# Autodesk Inventor assembly: Крейцкопфф
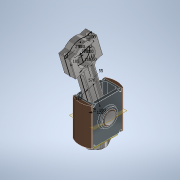
[picture p0: Inventor's stored thumbnail of the model, 180x180]
Saved by Autodesk Inventor 2021 (Build 250183000, 183)
## iProperties
Created: 2020-11-30
Part Number: Крейцкопфф
Document SubType Name: Assembly
Designer: Тимоха
Author: Тимоха
## Documents named in this file (17)
- C:\Users\Тимоха\Desktop\КР Компрессор\compressor\Крейцкопфф.iam
- C:\Users\Тимоха\Desktop\КР Компрессор\compressor\Втулка палец шатун.ipt
- C:\Users\Тимоха\Desktop\КР Компрессор\compressor\Втулка под палец.ipt
- C:\Users\Тимоха\Desktop\КР Компрессор\compressor\Крейцкопф.ipt
- C:\Users\Тимоха\Desktop\КР Компрессор\compressor\Шатун.ipt
- C:\Users\Тимоха\Desktop\КР Компрессор\compressor\Втулка под палец_MIR.ipt
- C:\Users\Тимоха\Desktop\КР Компрессор\compressor\Палец.ipt
- C:\Users\Тимоха\Desktop\КР Компрессор\compressor\Фланецгайка.ipt
- C:\Users\Тимоха\Desktop\КР Компрессор\compressor\Башмак.ipt
- C:\Users\Тимоха\Desktop\КР Компрессор\compressor\Башмак_MIR.ipt
- C:\Users\Тимоха\Desktop\КР Компрессор\compressor\Гайка шток.ipt
- C:\Users\Тимоха\Desktop\КР Компрессор\compressor\Прокладка крейцкопф.ipt
- C:\Users\Тимоха\Documents\Inventor\Content Center Files\R2021\ru-RU\GOST 8878-93\Винт M6-6gx25 ГОСТ 8878-93.ipt
- C:\Users\Тимоха\Documents\Inventor\Content Center Files\R2021\ru-RU\GOST 11371-78  A\Шайба 8 ГОСТ 11371-78.ipt
- C:\Users\Тимоха\Documents\Inventor\Content Center Files\R2021\ru-RU\Nut GOST 15524-70\Гайка M6-6H ГОСТ 15524-70.ipt
- C:\Users\Тимоха\Desktop\КР Компрессор\compressor\Стопорное кольцо.ipt
- C:\Users\Тимоха\Desktop\КР Компрессор\compressor\Стопорное кольцо_MIR.ipt
## Components (37 placed, 16 different names)
1. Втулка палец шатун:1 — Жесткий:2, С поворотом:1
2. Втулка под палец:1 — Жесткий:1
3. Крейцкопф:1 — Жесткий:1, Жесткий:5, Жесткий:6, Заподлицо:1, Заподлицо:2, Жесткий:8, Заподлицо:3
4. Втулка под палец_MIR:1 — Жесткий:2, Жесткий:5, Жесткий:20
5. Башмак:1 — Жесткий:6, Жесткий:7
6. Башмак_MIR:1
7. Прокладка крейцкопф:1 — Заподлицо:1, Заподлицо:2, Жесткий:18
8. Винт ГОСТ 8878-93 M6 x 25:1 — Жесткий:7
9. Шайба  ГОСТ 11371-78 8,4:1 — Жесткий:8, Жесткий:9
10. Гайка ГОСТ 15524-70 M6:1 — Жесткий:9
11. Винт ГОСТ 8878-93 M6 x 25:3
12. Шайба  ГОСТ 11371-78 8,4:3 — Жесткий:11
13. Гайка ГОСТ 15524-70 M6:3 — Жесткий:11
14. Винт ГОСТ 8878-93 M6 x 25:4
15. Шайба  ГОСТ 11371-78 8,4:4 — Жесткий:12
16. Гайка ГОСТ 15524-70 M6:4 — Жесткий:12
17. Винт ГОСТ 8878-93 M6 x 25:5
18. Шайба  ГОСТ 11371-78 8,4:5 — Жесткий:13
19. Гайка ГОСТ 15524-70 M6:5 — Жесткий:13
20. Винт ГОСТ 8878-93 M6 x 25:6
21. Шайба  ГОСТ 11371-78 8,4:6 — Жесткий:14
22. Гайка ГОСТ 15524-70 M6:6 — Жесткий:14
23. Винт ГОСТ 8878-93 M6 x 25:7
24. Шайба  ГОСТ 11371-78 8,4:7 — Жесткий:15
25. Гайка ГОСТ 15524-70 M6:7 — Жесткий:15
26. Винт ГОСТ 8878-93 M6 x 25:8
27. Шайба  ГОСТ 11371-78 8,4:8 — Жесткий:16
28. Гайка ГОСТ 15524-70 M6:8 — Жесткий:16
29. Винт ГОСТ 8878-93 M6 x 25:9
30. Шайба  ГОСТ 11371-78 8,4:9 — Жесткий:17
31. Гайка ГОСТ 15524-70 M6:9 — Жесткий:17
32. Гайка шток:1 — Жесткий:19
33. Фланецгайка:1 — Жесткий:18, Жесткий:19, Совмещение:1, Совмещение:2
34. Палец:1 — Жесткий:20, Заподлицо:4, Заподлицо:5
35. Стопорное кольцо:1 — Заподлицо:4, Заподлицо:5
36. Стопорное кольцо_MIR:1
37. Шатун:1 — С поворотом:1, Угол:1
## Relationships (26: WeldJoint 17, Flush 5, Mate 2, RevoluteJoint 1, Angle 1)
- Жесткий:1 [WeldJoint]: Втулка под палец:1 ↔ Крейцкопф:1
- Жесткий:2 [WeldJoint]: Втулка палец шатун:1 ↔ Втулка под палец_MIR:1
- Жесткий:5 [WeldJoint]: Крейцкопф:1 ↔ Втулка под палец_MIR:1
- Жесткий:6 [WeldJoint]: Крейцкопф:1 ↔ Башмак:1
- Заподлицо:1 [Flush]: Крейцкопф:1 ↔ Прокладка крейцкопф:1
- Заподлицо:2 [Flush]: Крейцкопф:1 ↔ Прокладка крейцкопф:1
- Жесткий:7 [WeldJoint]: Башмак:1 ↔ Винт ГОСТ 8878-93 M6 x 25:1
- Жесткий:8 [WeldJoint]: Крейцкопф:1 ↔ Шайба  ГОСТ 11371-78 8,4:1
- Жесткий:9 [WeldJoint]: Шайба  ГОСТ 11371-78 8,4:1 ↔ Гайка ГОСТ 15524-70 M6:1
- Жесткий:11 [WeldJoint]: Шайба  ГОСТ 11371-78 8,4:3 ↔ Гайка ГОСТ 15524-70 M6:3
- Жесткий:12 [WeldJoint]: Шайба  ГОСТ 11371-78 8,4:4 ↔ Гайка ГОСТ 15524-70 M6:4
- Жесткий:13 [WeldJoint]: Шайба  ГОСТ 11371-78 8,4:5 ↔ Гайка ГОСТ 15524-70 M6:5
- Заподлицо:3 [Flush] (-175 mm): Крейцкопф:1
- Жесткий:14 [WeldJoint]: Шайба  ГОСТ 11371-78 8,4:6 ↔ Гайка ГОСТ 15524-70 M6:6
- Жесткий:15 [WeldJoint]: Шайба  ГОСТ 11371-78 8,4:7 ↔ Гайка ГОСТ 15524-70 M6:7
- Жесткий:16 [WeldJoint]: Шайба  ГОСТ 11371-78 8,4:8 ↔ Гайка ГОСТ 15524-70 M6:8
- Жесткий:17 [WeldJoint]: Шайба  ГОСТ 11371-78 8,4:9 ↔ Гайка ГОСТ 15524-70 M6:9
- Жесткий:18 [WeldJoint]: Прокладка крейцкопф:1 ↔ Фланецгайка:1
- Жесткий:19 [WeldJoint]: Гайка шток:1 ↔ Фланецгайка:1
- Жесткий:20 [WeldJoint]: Втулка под палец_MIR:1 ↔ Палец:1
- Заподлицо:4 [Flush]: Палец:1 ↔ Стопорное кольцо:1
- Заподлицо:5 [Flush]: Палец:1 ↔ Стопорное кольцо:1
- Совмещение:1 [Mate]: Фланецгайка:1
- Совмещение:2 [Mate]: Фланецгайка:1
- С поворотом:1 [RevoluteJoint]: Втулка палец шатун:1 ↔ Шатун:1
- Угол:1 [Angle] (168.5 deg): Шатун:1
